# Autodesk Inventor assembly: test-model-2025b
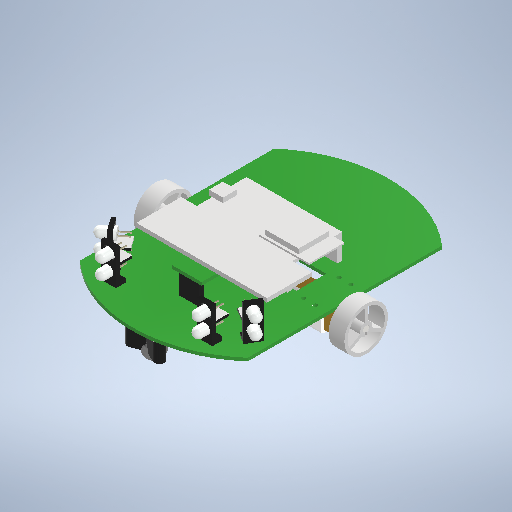
[picture p0: Inventor's stored thumbnail of the model, 512x512]
Saved by Autodesk Inventor 2025.3 (Build 293356000, 356)
## iProperties
Created: 2025-05-29
Part Number: test-model-2025b
Document SubType Name: Assembly
Designer: yamashita1
Author: yamashita1
## Documents named in this file (8)
- G:\マイドライブ\project\micro-mouse\3D-Model\test-model-2025b.iam
- G:\マイドライブ\project\micro-mouse\3D-Model\BaseBoard1.ipt
- G:\マイドライブ\project\micro-mouse\3D-Model\N20withBracket.iam
- G:\マイドライブ\project\micro-mouse\3D-Model\BallCaster-H16.ipt
- G:\マイドライブ\project\micro-mouse\3D-Model\D-Shaft_Wheel3.ipt
- G:\マイドライブ\project\micro-mouse\3D-Model\ESP32-DevKitC.ipt
- G:\マイドライブ\project\micro-mouse\3D-Model\AE-AQM1602A.ipt
- G:\マイドライブ\project\micro-mouse\3D-Model\Photo-Sensor.iam
## Components (13 placed, 7 different names)
1. BaseBoard1:1 — メイト:1, メイト:2, メイト:3, メイト:4, メイト:8, メイト:9, メイト:10, メイト:11, メイト:12, メイト:13, メイト:14, メイト:15
2. N20withBracket:1 [sub-assembly] — メイト:1, メイト:6, メイト:7, メイト:9
3. N20withBracket:2 [sub-assembly] — メイト:2, メイト:5, メイト:10
4. BallCaster-H16:1 — メイト:3
5. BallCaster-H16:2 — メイト:4
6. D-Shaft_Wheel3:1 — メイト:5
7. D-Shaft_Wheel3:2 — メイト:6, メイト:7
8. ESP32-DevKitC:1 — メイト:8
9. AE-AQM1602A:1 — メイト:11
10. Photo-Sensor:1 [sub-assembly] — メイト:12
11. Photo-Sensor:2 [sub-assembly] — メイト:13
12. Photo-Sensor:3 [sub-assembly] — メイト:14
13. Photo-Sensor:4 [sub-assembly] — メイト:15
## Relationships (15: Mate 15)
- メイト:1 [Mate]: BaseBoard1:1 ↔ N20withBracket:1
- メイト:2 [Mate]: BaseBoard1:1 ↔ N20withBracket:2
- メイト:3 [Mate]: BaseBoard1:1 ↔ BallCaster-H16:1
- メイト:4 [Mate]: BaseBoard1:1 ↔ BallCaster-H16:2
- メイト:5 [Mate]: N20withBracket:2 ↔ D-Shaft_Wheel3:1
- メイト:6 [Mate]: N20withBracket:1 ↔ D-Shaft_Wheel3:2
- メイト:7 [Mate]: N20withBracket:1 ↔ D-Shaft_Wheel3:2
- メイト:8 [Mate]: BaseBoard1:1 ↔ ESP32-DevKitC:1
- メイト:9 [Mate]: BaseBoard1:1 ↔ N20withBracket:1
- メイト:10 [Mate]: BaseBoard1:1 ↔ N20withBracket:2
- メイト:11 [Mate]: BaseBoard1:1 ↔ AE-AQM1602A:1
- メイト:12 [Mate]: BaseBoard1:1 ↔ Photo-Sensor:1
- メイト:13 [Mate]: BaseBoard1:1 ↔ Photo-Sensor:2
- メイト:14 [Mate]: BaseBoard1:1 ↔ Photo-Sensor:3
- メイト:15 [Mate]: BaseBoard1:1 ↔ Photo-Sensor:4
